# Autodesk Inventor assembly: AngelBox
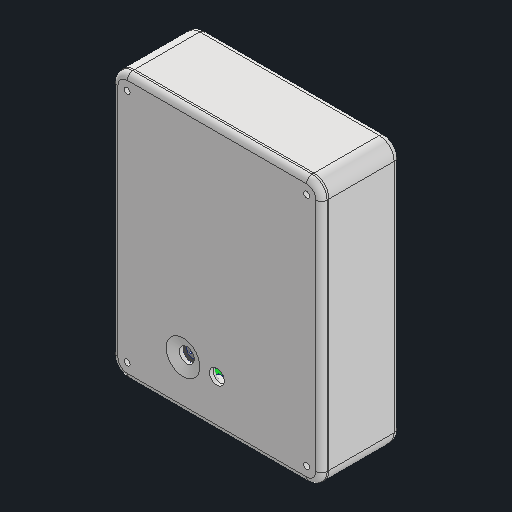
[picture p0: Inventor's stored thumbnail of the model, 512x512]
Saved by Autodesk Inventor 2026.2 (Build 302298000, 298)
## iProperties
Created: 2026-02-21
Part Number: AngelBox
Document SubType Name: Assembly
Designer: niuke
Author: niuke
## Documents named in this file (4)
- C:\Users\niuke\Documents\GitHub\angel-box\CAD\AngelBox.iam
- C:\Users\niuke\Documents\GitHub\angel-box\CAD\Parts\Jetson Nano 2GB\Jetson Nano 2GB.iam
- C:\Users\niuke\Documents\GitHub\angel-box\CAD\Housing.ipt
- C:\Users\niuke\Documents\GitHub\angel-box\CAD\LidAssem.iam
## Components (3 placed, 3 different names)
1. Jetson Nano 2GB:1 [sub-assembly] — Flush:1, Flush:2, Flush:3
2. Housing:1 — Flush:1, Flush:3, Mate:1, Mate:2, Mate:3
3. LidAssem:1 [sub-assembly] — Mate:1, Mate:2, Mate:3
## Relationships (6: Flush 3, Mate 3)
- Flush:1: Jetson Nano 2GB:1 ↔ Housing:1
- Flush:2 (4 mm): Jetson Nano 2GB:1
- Flush:3 (1.6002 mm): Jetson Nano 2GB:1 ↔ Housing:1
- Mate:1: Housing:1 ↔ LidAssem:1
- Mate:2: Housing:1 ↔ LidAssem:1
- Mate:3: Housing:1 ↔ LidAssem:1
